# Autodesk Inventor assembly: montagem
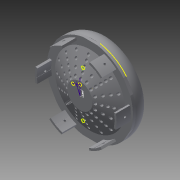
[picture p0: Inventor's stored thumbnail of the model, 180x180]
Saved by Autodesk Inventor 2015 (Build 190159000, 159)
## iProperties
Created: 2019-09-28
Part Number: montagem
Document SubType Name: Assembly
Designer: gabri
Author: gabri
## Documents named in this file (6)
- C:\Users\gabri\Documents\Inventor\cansat-3d\montagem.iam
- C:\Users\gabri\Documents\Inventor\cansat-3d\data_logger.ipt
- C:\Users\gabri\Documents\Inventor\cansat-3d\cup.ipt
- C:\Users\gabri\Documents\Inventor\cansat-3d\base.ipt
- C:\Users\gabri\Documents\Inventor\cansat-3d\corpo.ipt
- C:\Users\gabri\Documents\Inventor\cansat-3d\nose.ipt
## Components (5 placed, 5 different names)
1. cup:1 — Mate:1, Mate:2, Mate:3
2. base:1 — Flush:1, Flush:2
3. corpo:1 — Flush:2, Flush:3
4. nose:1 — Flush:3
5. data_logger:1 — Mate:1, Mate:2, Mate:3, Flush:1
## Relationships (6: Mate 3, Flush 3)
- Mate:1: cup:1 ↔ data_logger:1
- Mate:2: cup:1 ↔ data_logger:1
- Mate:3: cup:1 ↔ data_logger:1
- Flush:1: base:1 ↔ data_logger:1
- Flush:2: base:1 ↔ corpo:1
- Flush:3: corpo:1 ↔ nose:1
